# Autodesk Inventor assembly: FirstAssembly
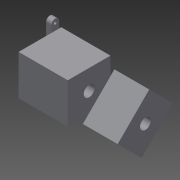
[picture p0: Inventor's stored thumbnail of the model, 180x180]
Saved by Autodesk Inventor 2014 SP1 (Build 180222100, 222)
## iProperties
Created: 2014-03-23
Part Number: FirstAssembly
Document SubType Name: Assembly
Designer: Mark
Author: Mark
## Documents named in this file (4)
- F:\Users\Mark\Documents\inventor\GitHub\FirstAssembly.iam
- F:\Users\Mark\Documents\Inventor\GitHub\BOX.ipt
- F:\Users\Mark\Documents\Inventor\GitHub\TEST.ipt
- F:\Users\Mark\Documents\Inventor\GitHub\BOX_WITH_HOLE.ipt
## Components (3 placed, 3 different names)
1. TEST:1 — Rotational:1
2. BOX:1 — Rotational:2, Rotational:1
3. BOX_WITH_HOLE:1 — Rotational:2
## Relationships (2: RevoluteJoint 2)
- Rotational:1 [RevoluteJoint]: TEST:1 ↔ BOX:1
- Rotational:2 [RevoluteJoint] (-12.7 mm): BOX:1 ↔ BOX_WITH_HOLE:1
## Named parameters: d3_d0 = -12.7 mm
